# Autodesk Inventor assembly: PCB_LEPF
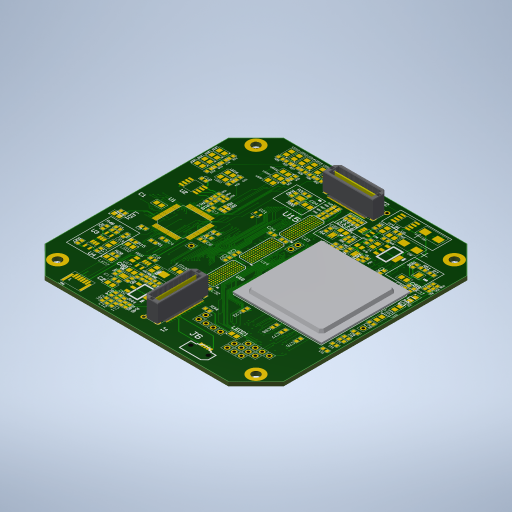
[picture p0: Inventor's stored thumbnail of the model, 512x512]
Saved by Autodesk Inventor 2023 (Build 270158000, 158)
## iProperties
Created: 2011-10-12
Part Number: PCB_LEPF
Document SubType Name: Assembly
Designer: Robert Davis
Description: EXPERIMENT #1 PCB
Mass: 35.2633 g
Surface Area: 354.09 cm^2
Volume: 16.1818 cm^3
Density: 2.17919 g/cm^3
Author: Robert Davis
## Documents named in this file (6)
- E:\Dropbox\AMSAT\CAD_backup_frequent_files_20200629\PCB_LEPF.iam
- E:\Dropbox\AMSAT\CAD_backup_frequent_files_20200629\Samtec_QSH-030-01-L-D-A.ipt
- E:\Dropbox\AMSAT\CAD_backup_frequent_files_20200629\Samtec_QTH-030-02-L-D-A.ipt
- E:\Dropbox\AMSAT\CAD_backup_frequent_files_20200629\Exp1_extramass.ipt
- E:\Dropbox\AMSAT\CAD_backup_frequent_files_20200629\PCB_LEPF.ipt
- E:\Dropbox\AMSAT\CAD_backup_frequent_files_20200629\REM_SRAM_BGA.ipt
## Components (7 placed, 5 different names)
1. PCB_LEPF:1 — Mate:3, Mate:4, Angle:3, Mate:1, Mate:2, Angle:4, Mate:5, Mate:7, Tangent:1
2. Samtec_QTH-030-02-L-D-A:1 — Mate:1, Mate:2, Angle:4
3. Samtec_QSH-030-01-L-D-A:1 — Mate:3, Mate:4, Angle:3
4. Samtec_QTH-030-02-L-D-A:2 — Mate:5, Mate:6
5. Exp1_extramass:1 — Flush:2, Flush:3, Flush:4
6. Samtec_QSH-030-01-L-D-A:2 — Mate:7, Mate:8, Mate:9
7. REM_SRAM_BGA:1 — Tangent:1, Mate:10, Mate:11
## Relationships (18: Mate 11, Flush 4, Angle 2, Tangent 1)
- Mate:3: PCB_LEPF:1 ↔ Samtec_QSH-030-01-L-D-A:1
- Mate:4: PCB_LEPF:1 ↔ Samtec_QSH-030-01-L-D-A:1
- Angle:3 (180 deg): PCB_LEPF:1 ↔ Samtec_QSH-030-01-L-D-A:1
- Mate:1: PCB_LEPF:1 ↔ Samtec_QTH-030-02-L-D-A:1
- Mate:2: PCB_LEPF:1 ↔ Samtec_QTH-030-02-L-D-A:1
- Angle:4 (180 deg): PCB_LEPF:1 ↔ Samtec_QTH-030-02-L-D-A:1
- Mate:5: PCB_LEPF:1 ↔ Samtec_QTH-030-02-L-D-A:2
- [Flush]: Samtec_QTH-030-02-L-D-A:2
- Mate:6 (39.5 mm): Samtec_QTH-030-02-L-D-A:2
- Flush:2: Exp1_extramass:1
- Flush:3: Exp1_extramass:1
- Flush:4: Exp1_extramass:1
- Mate:7: PCB_LEPF:1 ↔ Samtec_QSH-030-01-L-D-A:2
- Mate:8: Samtec_QSH-030-01-L-D-A:2
- Mate:9 (39.5 mm): Samtec_QSH-030-01-L-D-A:2
- Tangent:1: PCB_LEPF:1 ↔ REM_SRAM_BGA:1
- Mate:10 (25 mm): REM_SRAM_BGA:1
- Mate:11 (1 mm): REM_SRAM_BGA:1
